# Autodesk Inventor assembly: Elevator System Master
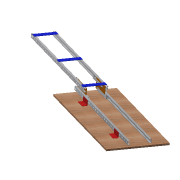
[picture p0: Inventor's stored thumbnail of the model, 180x180]
Saved by Autodesk Inventor 2015 (Build 190159000, 159)
## iProperties
Created: 2014-09-27
Part Number: Elevator System Master
Document SubType Name: Assembly
Designer: Peter
Author: Peter
## Documents named in this file (9)
- T:\FILES\Inventor 2015 Projects\Elevator Version 2\Elevator System Master.iam
- T:\FILES\Inventor 2015 Projects\Elevator Version 2\Plywood.ipt
- T:\FILES\Inventor 2015 Projects\Elevator Version 2\MountingBracket.ipt
- T:\FILES\Inventor 2015 Projects\Elevator Version 2\Frc Chassis 2014\Unistrut 4ft.ipt
- T:\FILES\Inventor 2015 Projects\Elevator Version 2\Frc Chassis 2014\Car Assembly - Solo.iam
- T:\FILES\Inventor 2015 Projects\Elevator Version 2\MountingBracket_MIR.ipt
- T:\FILES\Inventor 2015 Projects\Elevator Version 2\Frc Chassis 2014\Unistrut 4ft_MIR.ipt
- T:\FILES\Inventor 2015 Projects\Elevator Version 2\Frc Chassis 2014\Car Assembly - Solo_MIR.iam
- T:\FILES\Inventor 2015 Projects\Elevator Version 2\Frc Chassis 2014\cross brace.ipt
## Components (16 placed, 8 different names)
1. Plywood:1 — Mate:1, Mate:2, Flush:2, Flush:3, Flush:4, Mate:4, Flush:5
2. MountingBracket:1 — Mate:2, Flush:1, Flush:3, Flush:4, Mate:3
3. MountingBracket:2 — Mate:1, Flush:1, Flush:2
4. Unistrut 4ft:1 — Mate:3, Mate:4, Flush:5, Mate:5, Mate:6, Flush:6, Flush:7, Flush:9, Flush:17, Flush:18
5. Car Assembly - Solo:1 [sub-assembly] — Mate:5, Mate:6, Flush:8
6. Unistrut 4ft:2 — Flush:7, Flush:8, Flush:10, Mate:16, Mate:17, Flush:16, Flush:19, Flush:22
7. Car Assembly - Solo:2 [sub-assembly] — Flush:6, Flush:9
8. MountingBracket_MIR:1 — Flush:11, Mate:9
9. MountingBracket_MIR:2 — Flush:11
10. Unistrut 4ft_MIR:1 — Mate:9, Mate:10, Mate:11, Flush:13, Flush:14, Flush:15, Flush:24
11. Car Assembly - Solo_MIR:1 [sub-assembly] — Mate:10, Mate:11, Flush:12, Flush:24
12. Unistrut 4ft_MIR:2 — Flush:12, Flush:13, Mate:12, Mate:13, Mate:14, Mate:15, Flush:20, Flush:21, Flush:23
13. Car Assembly - Solo_MIR:2 [sub-assembly] — Flush:14, Flush:15, Mate:12, Mate:13
14. cross brace:1 — Mate:16, Flush:18, Flush:20
15. cross brace:2 — Mate:15, Flush:16, Flush:19, Flush:22, Flush:23
16. cross brace:3 — Mate:17, Flush:17, Flush:21
## Relationships (41: Flush 24, Mate 17)
- Mate:1: Plywood:1 ↔ MountingBracket:2
- Mate:2: Plywood:1 ↔ MountingBracket:1
- Flush:1: MountingBracket:1 ↔ MountingBracket:2
- Flush:2 (-203.2 mm): Plywood:1 ↔ MountingBracket:2
- Flush:3 (203.2 mm): Plywood:1 ↔ MountingBracket:1
- Flush:4 (127 mm): Plywood:1 ↔ MountingBracket:1
- Mate:3: MountingBracket:1 ↔ Unistrut 4ft:1
- Mate:4 (19.05 mm): Plywood:1 ↔ Unistrut 4ft:1
- Flush:5: Plywood:1 ↔ Unistrut 4ft:1
- Mate:5 (2.8702 mm): Unistrut 4ft:1 ↔ Car Assembly - Solo:1
- Mate:6 (2.286 mm): Unistrut 4ft:1 ↔ Car Assembly - Solo:1
- [Mate] (2.8702 mm): Unistrut 4ft:2 ↔ Car Assembly - Solo:2
- [Mate] (2.286 mm): Unistrut 4ft:2 ↔ Car Assembly - Solo:2
- Flush:6 (2.286 mm): Unistrut 4ft:1 ↔ Car Assembly - Solo:2
- Flush:7: Unistrut 4ft:1 ↔ Unistrut 4ft:2
- Flush:8: Car Assembly - Solo:1 ↔ Unistrut 4ft:2
- Flush:9: Unistrut 4ft:1 ↔ Car Assembly - Solo:2
- Flush:10 (93.6625 mm): Unistrut 4ft:2
- Flush:11: MountingBracket_MIR:1 ↔ MountingBracket_MIR:2
- Mate:9: MountingBracket_MIR:1 ↔ Unistrut 4ft_MIR:1
- Mate:10 (2.286 mm): Unistrut 4ft_MIR:1 ↔ Car Assembly - Solo_MIR:1
- Mate:11 (2.8702 mm): Unistrut 4ft_MIR:1 ↔ Car Assembly - Solo_MIR:1
- Flush:12: Car Assembly - Solo_MIR:1 ↔ Unistrut 4ft_MIR:2
- Flush:13: Unistrut 4ft_MIR:1 ↔ Unistrut 4ft_MIR:2
- Flush:14: Unistrut 4ft_MIR:1 ↔ Car Assembly - Solo_MIR:2
- Flush:15 (2.286 mm): Unistrut 4ft_MIR:1 ↔ Car Assembly - Solo_MIR:2
- Mate:12 (2.286 mm): Unistrut 4ft_MIR:2 ↔ Car Assembly - Solo_MIR:2
- Mate:13 (2.8702 mm): Unistrut 4ft_MIR:2 ↔ Car Assembly - Solo_MIR:2
- Mate:14 (93.6625 mm): Unistrut 4ft_MIR:2
- Mate:15: Unistrut 4ft_MIR:2 ↔ cross brace:2
- Mate:16: Unistrut 4ft:2 ↔ cross brace:1
- Mate:17: Unistrut 4ft:2 ↔ cross brace:3
- Flush:16: Unistrut 4ft:2 ↔ cross brace:2
- Flush:17: Unistrut 4ft:1 ↔ cross brace:3
- Flush:18: Unistrut 4ft:1 ↔ cross brace:1
- Flush:19 (25.4 mm): Unistrut 4ft:2 ↔ cross brace:2
- Flush:20 (25.4 mm): Unistrut 4ft_MIR:2 ↔ cross brace:1
- Flush:21 (-584.2 mm): Unistrut 4ft_MIR:2 ↔ cross brace:3
- Flush:22 (25.4 mm): Unistrut 4ft:2 ↔ cross brace:2
- Flush:23 (25.4 mm): Unistrut 4ft_MIR:2 ↔ cross brace:2
- Flush:24 (-431.8 mm): Unistrut 4ft_MIR:1 ↔ Car Assembly - Solo_MIR:1
## Named parameters: d19_d13 = 2.8702 mm, d20_d14 = 2.286 mm
